# Autodesk Inventor assembly: Rr.wing_cradle
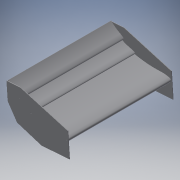
[picture p0: Inventor's stored thumbnail of the model, 180x180]
Saved by Autodesk Inventor 2018.2 (Build 222227000, 227)
## iProperties
Created: 2018-03-07
Part Number: Rr.wing_cradle
Material: 一般
Document SubType Name: Assembly
Designer: ku_sk
Author: ku_sk
## Documents named in this file (4)
- C:\Users\ku_sk\Documents\Inventor\Aero\KS-15\Rr.wing\cradle\parts\Rr.wing_cradle.iam
- C:\Users\ku_sk\Documents\Inventor\Aero\KS-15\Rr.wing\cradle\parts\main frap.ipt
- C:\Users\ku_sk\Documents\Inventor\Aero\KS-15\Rr.wing\cradle\parts\subflap.ipt
- C:\Users\ku_sk\Documents\Inventor\Aero\KS-15\Rr.wing\cradle\parts\endplate.ipt
## Components (5 placed, 3 different names)
1. main frap:1 — メイト:1, フラッシュ:1, メイト:2, メイト:3, メイト:4, メイト:5, 角度:1, 角度:2
2. subflap:1 — メイト:6, メイト:7, 角度:2, 角度:3
3. endplate:1 — メイト:3, メイト:4, フラッシュ:2, メイト:7, メイト:8, メイト:9
4. endplate:2 — メイト:2, メイト:5, フラッシュ:2, メイト:6
5. subflap:2 — メイト:8, メイト:9, 角度:3
## Relationships (14: Mate 9, Angle 3, Flush 2)
- メイト:1 [Mate]: main frap:1
- フラッシュ:1 [Flush]: main frap:1
- メイト:2 [Mate]: main frap:1 ↔ endplate:2
- メイト:3 [Mate]: main frap:1 ↔ endplate:1
- メイト:4 [Mate]: main frap:1 ↔ endplate:1
- メイト:5 [Mate]: main frap:1 ↔ endplate:2
- フラッシュ:2 [Flush]: endplate:1 ↔ endplate:2
- メイト:6 [Mate]: subflap:1 ↔ endplate:2
- メイト:7 [Mate]: subflap:1 ↔ endplate:1
- メイト:8 [Mate]: endplate:1 ↔ subflap:2
- メイト:9 [Mate]: endplate:1 ↔ subflap:2
- 角度:1 [Angle] (15 deg): main frap:1
- 角度:2 [Angle] (-15 deg): main frap:1 ↔ subflap:1
- 角度:3 [Angle] (-15 deg): subflap:1 ↔ subflap:2
